# Autodesk Inventor assembly: сборка основания
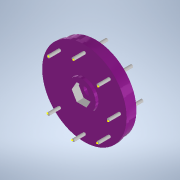
[picture p0: Inventor's stored thumbnail of the model, 180x180]
Saved by Autodesk Inventor 2022 (Build 260153000, 153)
## iProperties
Created: 2024-04-29
Part Number: сборка основания
Document SubType Name: Assembly
Designer: Pavel
Mass: 2.40614 g
Surface Area: 23.23 cm^2
Volume: 2.40614 cm^3
Density: 1 g/cm^3
Author: Pavel
## Documents named in this file (3)
- D:\BSUIR\KMEKES\сборка основания.iam
- D:\BSUIR\KMEKES\основание.ipt
- D:\BSUIR\KMEKES\штырь.ipt
## Components (8 placed, 2 different names)
1. основание:1 — Вставка:1
2. штырь:1 — Вставка:1
3. штырь:2
4. штырь:3
5. штырь:4
6. штырь:5
7. штырь:6
8. штырь:7
## Component patterns: (7 elements, first: штырь:1)
## Relationships (2: Flush 1, Insert 1)
- Заподлицо:1 [Flush] (1.75 mm)
- Вставка:1 [Insert]: основание:1 ↔ штырь:1
